# Autodesk Inventor assembly: установщик образцов 2
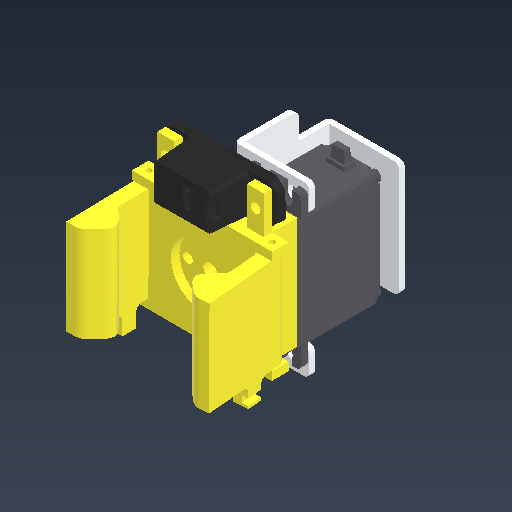
[picture p0: Inventor's stored thumbnail of the model, 512x512]
Saved by Autodesk Inventor 2025 (Build 290162000, 162)
## iProperties
Created: 2025-01-28
Part Number: установщик образцов 2
Document SubType Name: Assembly
Designer: GameHD
Author: GameHD
## Documents named in this file (7)
- C:\Users\GameHD\Desktop\phantom 16950\установщик образцов 2.iam
- C:\Users\GameHD\Desktop\phantom 16950\bratzahvatstp\bratzahvatstp.ipt
- C:\Users\GameHD\Desktop\phantom 16950\brat2zahvat\brat2zahvat.ipt
- C:\Users\GameHD\Desktop\phantom 16950\39060_txm-standard servo bracket\39060_txm-standard servo bracket_MIR1.ipt
- C:\Users\GameHD\Desktop\phantom 16950\2000-0025-0002\2000-0025-0002_MIR2.ipt
- C:\Users\GameHD\Desktop\phantom 16950\brat2zahvat\brat2zahvat_MIR.ipt
- C:\Users\GameHD\Downloads\Telegram Desktop\REV-31-1557\REV-31-1557.ipt
## Components (6 placed, 6 different names)
1. bratzahvatstp:1
2. brat2zahvat:1
3. 39060_txm-standard servo bracket_MIR1:1
4. 2000-0025-0002_MIR2:1
5. brat2zahvat_MIR:1
6. REV-31-1557:1
## Relationships (11: Mate 10, Flush 1)
- [Mate]: 39060_txm-standard servo bracket_MIR1:1 ↔ 2000-0025-0002_MIR2:1
- [Mate] (4.5 mm): 39060_txm-standard servo bracket_MIR1:1 ↔ 2000-0025-0002_MIR2:1
- [Flush] (2 mm): 39060_txm-standard servo bracket_MIR1:1 ↔ 2000-0025-0002_MIR2:1
- [Mate]: bratzahvatstp:1 ↔ 2000-0025-0002_MIR2:1
- [Mate]: bratzahvatstp:1 ↔ 2000-0025-0002_MIR2:1
- [Mate]: bratzahvatstp:1 ↔ brat2zahvat:1
- [Mate]: bratzahvatstp:1 ↔ brat2zahvat_MIR:1
- [Mate]: bratzahvatstp:1 ↔ brat2zahvat:1
- [Mate]: bratzahvatstp:1 ↔ brat2zahvat_MIR:1
- [Mate]: bratzahvatstp:1 ↔ REV-31-1557:1
- [Mate]: bratzahvatstp:1 ↔ REV-31-1557:1
## Named parameters: d500_d406 = 4.5 mm, d501_d407 = 2 mm, d502_d275 = 0 mm
